# Autodesk Inventor assembly: SolarPanel
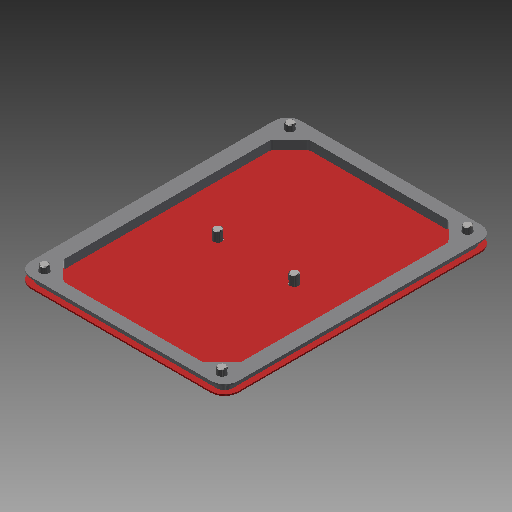
[picture p0: Inventor's stored thumbnail of the model, 512x512]
Saved by Autodesk Inventor 2018 (Build 220112000, 112)
## iProperties
Created: 2018-05-13
Part Number: SolarPanel
Document SubType Name: Assembly
Designer: Bradley
Author: Bradley
## Documents named in this file (6)
- D:\Users\Bradley\Documents\CougsInSpace\CougSat1-Hardware\CougSat1-PowerBoard\CADModel\Native\SolarPanel+Z.iam
- D:\Users\Bradley\Documents\CougsInSpace\CougSat1-Hardware\CougSat1-PowerBoard\CADModel\Native\SolarPanel_PCB.ipt
- D:\Users\Bradley\Documents\CougsInSpace\CougSat1-Hardware\CougSat1-PowerBoard\CADModel\Native\SolarPanel_CoilForm.ipt
- D:\Users\Bradley\Documents\CougsInSpace\Resources\ComponentModels\Electronics\SolarCell_UTJ.ipt
- D:\Users\Bradley\Documents\CougsInSpace\Resources\ComponentModels\Fasteners\Bolt_M3x0.35_6mm_BH.ipt
- D:\Users\Bradley\Documents\CougsInSpace\Resources\ComponentModels\Fasteners\Bolt_M3x0.35_4mm_BH.ipt
## Components (10 placed, 5 different names)
1. SolarPanel_CoilForm:1 — Insert:1, Insert:2
2. SolarPanel_PCB:1 — Insert:1, Insert:2, Insert:3, Insert:4, Insert:5, Insert:6, Insert:7, Insert:8, Mate:1, Mate:2
3. SolarCell_UTJ:1 — Mate:1, Flush:1, Flush:2
4. SolarCell_UTJ:2 — Mate:2, Mate:3, Mate:4
5. Bolt_M3x0.35_4mm_BH:1 — Insert:5
6. Bolt_M3x0.35_4mm_BH:2 — Insert:6
7. Bolt_M3x0.35_6mm_BH:3 — Insert:3
8. Bolt_M3x0.35_6mm_BH:4 — Insert:4
9. Bolt_M3x0.35_6mm_BH:1 — Insert:7
10. Bolt_M3x0.35_6mm_BH:2 — Insert:8
## Relationships (14: Insert 8, Mate 4, Flush 2)
- Insert:1: SolarPanel_CoilForm:1 ↔ SolarPanel_PCB:1
- Insert:2: SolarPanel_CoilForm:1 ↔ SolarPanel_PCB:1
- Insert:3: SolarPanel_PCB:1 ↔ Bolt_M3x0.35_6mm_BH:3
- Insert:4: SolarPanel_PCB:1 ↔ Bolt_M3x0.35_6mm_BH:4
- Insert:5: SolarPanel_PCB:1 ↔ Bolt_M3x0.35_4mm_BH:1
- Insert:6: SolarPanel_PCB:1 ↔ Bolt_M3x0.35_4mm_BH:2
- Insert:7: SolarPanel_PCB:1 ↔ Bolt_M3x0.35_6mm_BH:1
- Insert:8: SolarPanel_PCB:1 ↔ Bolt_M3x0.35_6mm_BH:2
- Mate:1: SolarPanel_PCB:1 ↔ SolarCell_UTJ:1
- Mate:2: SolarPanel_PCB:1 ↔ SolarCell_UTJ:2
- Flush:1: SolarCell_UTJ:1
- Mate:3: SolarCell_UTJ:2
- Mate:4 (5 mm): SolarCell_UTJ:2
- Flush:2 (5 mm): SolarCell_UTJ:1
